# Autodesk Inventor assembly: Zespół1
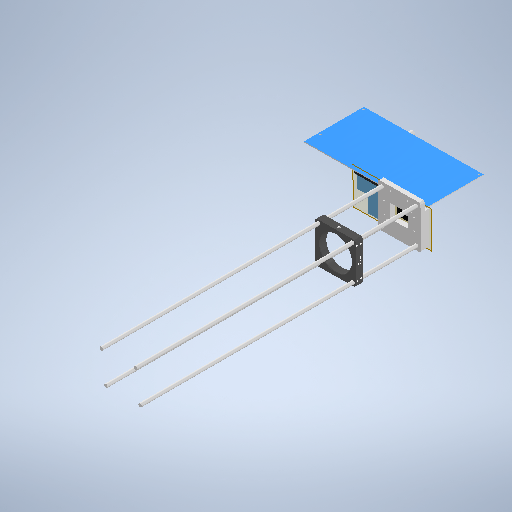
[picture p0: Inventor's stored thumbnail of the model, 512x512]
Saved by Autodesk Inventor 2025.1 (Build 291241000, 241)
## iProperties
Created: 2024-10-25
Part Number: Zespół1
Document SubType Name: Assembly
Designer: PC
Author: PC
## Documents named in this file (4)
- C:\Users\PC\Desktop\fotolito_czesci\nowe\Zespół1.iam
- C:\Users\PC\Desktop\fotolito_czesci\nowe\plyta_dmd.iam
- C:\Users\PC\Desktop\fotolito_czesci\rod.ipt
- C:\Users\PC\Desktop\fotolito_czesci\LCP09-Solidworks.ipt
## Components (6 placed, 3 different names)
1. plyta_dmd:1 [sub-assembly] — Zestawiające:1, Zestawiające:2, Zestawiające:3, Zestawiające:4, Zestawiające:5, Zestawiające:6, Równoległe:1, Równoległe:2, Kątowe:1
2. rod:1 — Zestawiające:1, Równoległe:1, Zestawiające:7
3. rod:2 — Zestawiające:2, Zestawiające:6
4. rod:3 — Zestawiające:3, Zestawiające:5
5. rod:4 — Zestawiające:4, Równoległe:2
6. LCP09-Solidworks:1 — Zestawiające:7, Kątowe:1
## Relationships (10: Mate 7, Flush 2, Angle 1)
- Zestawiające:1 [Mate]: plyta_dmd:1 ↔ rod:1
- Zestawiające:2 [Mate]: plyta_dmd:1 ↔ rod:2
- Zestawiające:3 [Mate]: plyta_dmd:1 ↔ rod:3
- Zestawiające:4 [Mate]: plyta_dmd:1 ↔ rod:4
- Zestawiające:5 [Mate]: plyta_dmd:1 ↔ rod:3
- Zestawiające:6 [Mate]: plyta_dmd:1 ↔ rod:2
- Równoległe:1 [Flush]: plyta_dmd:1 ↔ rod:1
- Równoległe:2 [Flush]: plyta_dmd:1 ↔ rod:4
- Zestawiające:7 [Mate]: rod:1 ↔ LCP09-Solidworks:1
- Kątowe:1 [Angle] (0 deg): plyta_dmd:1 ↔ LCP09-Solidworks:1
